# Autodesk Inventor assembly: Delrin Mini V-Wheel
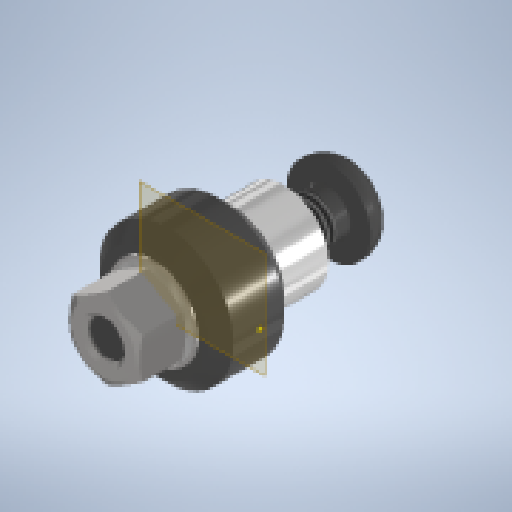
[picture p0: Inventor's stored thumbnail of the model, 512x512]
Saved by Autodesk Inventor 2024.3 (Build 283343000, 343)
## iProperties
Created: 2016-10-15
Part Number: Delrin Mini V-Wheel
Material: Типовые
Document SubType Name: Assembly
Designer: skhalipa
Author: skhalipa
## Documents named in this file (7)
- C:\Users\Nada\OneDrive - Faculty of Engineering Ain Shams University\Desktop\Modeling model\Delrin Mini V-Wheel.iam
- C:\Users\Nada\OneDrive - Faculty of Engineering Ain Shams University\Desktop\Modeling model\Mini V-Wheel 1523.ipt
- C:\Users\Nada\OneDrive - Faculty of Engineering Ain Shams University\Desktop\Modeling model\MR105ZZ Bearing.ipt
- C:\Users\Nada\OneDrive - Faculty of Engineering Ain Shams University\Desktop\Modeling model\Nut M5 GOST 15526-70.ipt
- C:\Users\Nada\OneDrive - Faculty of Engineering Ain Shams University\Desktop\Modeling model\Precision Shim 1mm.ipt
- C:\Users\Nada\OneDrive - Faculty of Engineering Ain Shams University\Desktop\Modeling model\Screw M5x25 GOST 28963-91.ipt
- C:\Users\Nada\OneDrive - Faculty of Engineering Ain Shams University\Desktop\Modeling model\Aluminum Spacer 6mm.ipt
## Components (7 placed, 6 different names)
1. Mini V-Wheel 1523:1 — Вставка:2, Вставка:3, Вставка:4
2. MR105ZZ Bearing:1 — Вставка:3, Вставка:6
3. Гайка ГОСТ 15526-70 M5:1 — Вставка:6
4. Precision Shim 1mm:1 — Вставка:2
5. Винт ГОСТ 28963-91 M5x25:1 — Вставка:1
6. Aluminum Spacer 6mm:1 — Вставка:1, Вставка:5
7. MR105ZZ Bearing:2 — Вставка:4, Вставка:5
## Relationships (6: Insert 6)
- Вставка:1 [Insert] (5 mm): Винт ГОСТ 28963-91 M5x25:1 ↔ Aluminum Spacer 6mm:1
- Вставка:2 [Insert]: Mini V-Wheel 1523:1 ↔ Precision Shim 1mm:1
- Вставка:3 [Insert]: Mini V-Wheel 1523:1 ↔ MR105ZZ Bearing:1
- Вставка:4 [Insert]: Mini V-Wheel 1523:1 ↔ MR105ZZ Bearing:2
- Вставка:5 [Insert]: Aluminum Spacer 6mm:1 ↔ MR105ZZ Bearing:2
- Вставка:6 [Insert]: MR105ZZ Bearing:1 ↔ Гайка ГОСТ 15526-70 M5:1
